# Autodesk Inventor assembly: shield_flautista
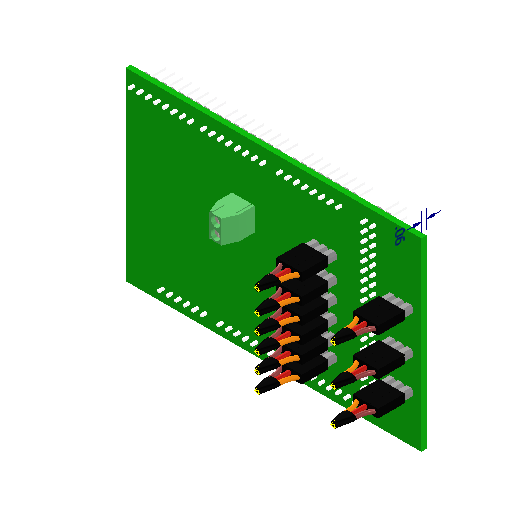
[picture p0: Inventor's stored thumbnail of the model, 512x512]
Saved by Autodesk Inventor 2022 (Build 260153000, 153)
## iProperties
Created: 2022-11-19
Part Number: shield_flautista
Document SubType Name: Assembly
Designer: Administrator
Title: shield_flautista v5
Author: Administrator
## Documents named in this file (6)
- C:\Users\ferna\Downloads\shield_flautista (1)\shield_flautista.iam
- C:\Users\ferna\Downloads\shield_flautista (1)\Board.ipt
- C:\Users\ferna\Downloads\shield_flautista (1)\Packages.iam
- C:\Users\ferna\Downloads\shield_flautista (1)\TERMINAL-BLOCK-2-PIN-3.5MM-LONG-PAD.ipt
- C:\Users\ferna\Downloads\shield_flautista (1)\1X01.ipt
- C:\Users\ferna\Documents\Bocas\Prototipo_09\arduino\concector_servos.ipt
## Components (94 placed, 5 different names)
1. Board:1 — Mate:1, Mate:2, Flush:1, Mate:3, Mate:4, Flush:2, Mate:7, Mate:8, Mate:9, Mate:10, Mate:11, Mate:12, Flush:3, Mate:13, Flush:4
2. Packages:1 [sub-assembly] — Mate:14, Flush:5, Flush:6, Flush:7, Mate:15, Flush:8, Flush:9, Mate:16, Flush:10, Flush:11, Mate:17, Flush:12, Flush:13, Mate:18, Flush:14, Flush:15, Mate:19, Flush:16, Flush:17, Mate:20, Flush:18, Flush:19, Mate:21, Flush:20, Flush:21, Mate:22, Flush:22
3. TERMINAL-BLOCK-2-PIN-3.5MM-LONG-PAD:1 — Mate:1, Mate:2, Flush:1
4. concector_servos:1 — Mate:14, Flush:5, Flush:6
5. concector_servos:2 — Flush:7, Mate:15, Flush:8
6. concector_servos:3 — Flush:9, Mate:16, Flush:10
7. concector_servos:4 — Flush:15, Mate:19, Flush:16
8. concector_servos:5 — Flush:13, Mate:18, Flush:14
9. concector_servos:6 — Flush:19, Mate:21, Flush:20
10. concector_servos:7 — Flush:11, Mate:17, Flush:12
11. concector_servos:8 — Flush:17, Mate:20, Flush:18
12. concector_servos:9 — Flush:21, Mate:22, Flush:22
13. 1X01:70 — Mate:11, Mate:12, Flush:3
14. 1X01:71
15. 1X01:72
16. 1X01:73
17. 1X01:74
18. 1X01:75
19. 1X01:6 — Mate:8, Mate:13, Flush:4
20. 1X01:76
21. 1X01:77
22. 1X01:78
23. 1X01:79
24. 1X01:80
25. 1X01:81
26. 1X01:82
27. 1X01:83
28. 1X01:84
29. 1X01:85
30. 1X01:86
31. 1X01:87
32. 1X01:88
33. 1X01:89
34. 1X01:90
35. 1X01:91
36. 1X01:92
37. 1X01:93
38. 1X01:94
39. 1X01:95
40. 1X01:96
41. 1X01:97
42. 1X01:98
43. 1X01:99
44. 1X01:100
45. 1X01:101
46. 1X01:102
47. 1X01:103
48. 1X01:104
49. 1X01:105
50. 1X01:106
51. 1X01:107
52. 1X01:108
53. 1X01:109
54. 1X01:110
55. 1X01:3 — Mate:7, Mate:9, Mate:10
56. 1X01:55
57. 1X01:56
58. 1X01:57
59. 1X01:58
60. 1X01:59
61. 1X01:60
62. 1X01:61
63. 1X01:62
64. 1X01:63
65. 1X01:64
66. 1X01:65
67. 1X01:66
68. 1X01:67
69. 1X01:68
70. 1X01:69
71. 1X01:1 — Mate:3, Mate:4, Flush:2
72. 1X01:8
73. 1X01:9
74. 1X01:10
75. 1X01:11
76. 1X01:12
77. 1X01:13
78. 1X01:14
79. 1X01:23
80. 1X01:24
81. 1X01:25
82. 1X01:26
83. 1X01:27
84. 1X01:28
85. 1X01:29
86. 1X01:30
87. 1X01:39
88. 1X01:40
89. 1X01:41
90. 1X01:42
91. 1X01:43
92. 1X01:44
93. 1X01:45
94. 1X01:46
## Component patterns: (2 elements), (2 elements), (6 elements, first: 1X01:70), (36 elements, first: 1X01:6), (2 elements), Component Pattern 2:2 (2 elements), (8 elements, first: 1X01:3), Component Pattern 4:2 (8 elements), (8 elements, first: 1X01:1), Component Pattern 1:2 (8 elements), Component Pattern 1:3 (8 elements)
## Relationships (42: Flush 22, Mate 20)
- Mate:1: Board:1 ↔ TERMINAL-BLOCK-2-PIN-3.5MM-LONG-PAD:1
- Mate:2 (-23.5 mm): Board:1 ↔ TERMINAL-BLOCK-2-PIN-3.5MM-LONG-PAD:1
- Flush:1 (-32 mm): Board:1 ↔ TERMINAL-BLOCK-2-PIN-3.5MM-LONG-PAD:1
- Mate:3: Board:1 ↔ 1X01:1
- Mate:4 (-4.75 mm): Board:1 ↔ 1X01:1
- Flush:2 (-22.85 mm): Board:1 ↔ 1X01:1
- Mate:7: Board:1 ↔ 1X01:3
- Mate:8: Board:1 ↔ 1X01:6
- Mate:9 (-5.05 mm): Board:1 ↔ 1X01:3
- Mate:10 (-19.35 mm): Board:1 ↔ 1X01:3
- Mate:11: Board:1 ↔ 1X01:70
- Mate:12 (-5.05 mm): Board:1 ↔ 1X01:70
- Flush:3 (-22.87 mm): Board:1 ↔ 1X01:70
- Mate:13 (-4.75 mm): Board:1 ↔ 1X01:6
- Flush:4 (12.68 mm): Board:1 ↔ 1X01:6
- Mate:14: Packages:1 ↔ concector_servos:1
- Flush:5: Packages:1 ↔ concector_servos:1
- Flush:6: Packages:1 ↔ concector_servos:1
- Flush:7: Packages:1 ↔ concector_servos:2
- Mate:15: Packages:1 ↔ concector_servos:2
- Flush:8: Packages:1 ↔ concector_servos:2
- Flush:9: Packages:1 ↔ concector_servos:3
- Mate:16: Packages:1 ↔ concector_servos:3
- Flush:10: Packages:1 ↔ concector_servos:3
- Flush:11: Packages:1 ↔ concector_servos:7
- Mate:17: Packages:1 ↔ concector_servos:7
- Flush:12: Packages:1 ↔ concector_servos:7
- Flush:13: Packages:1 ↔ concector_servos:5
- Mate:18: Packages:1 ↔ concector_servos:5
- Flush:14: Packages:1 ↔ concector_servos:5
- Flush:15: Packages:1 ↔ concector_servos:4
- Mate:19: Packages:1 ↔ concector_servos:4
- Flush:16: Packages:1 ↔ concector_servos:4
- Flush:17: Packages:1 ↔ concector_servos:8
- Mate:20: Packages:1 ↔ concector_servos:8
- Flush:18: Packages:1 ↔ concector_servos:8
- Flush:19: Packages:1 ↔ concector_servos:6
- Mate:21: Packages:1 ↔ concector_servos:6
- Flush:20: Packages:1 ↔ concector_servos:6
- Flush:21: Packages:1 ↔ concector_servos:9
- Mate:22: Packages:1 ↔ concector_servos:9
- Flush:22: Packages:1 ↔ concector_servos:9
